# Autodesk Inventor assembly: Flysky FS-iA6 Receiver
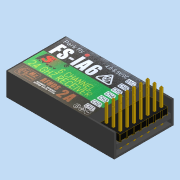
[picture p0: Inventor's stored thumbnail of the model, 180x180]
Saved by Autodesk Inventor 2022.3 (Build 263350030, 350C)
## iProperties
Created: 2022-09-05
Part Number: Flysky FS-iA6 Receiver
Document SubType Name: Assembly
Designer: admin
Author: admin
## Documents named in this file (3)
- C:\OneDrive\OneDrive - Personal\OneDrive\Documents\Inventor\BattleBot\Flysky FS-iA6 Receiver.iam
- C:\OneDrive\OneDrive - Personal\OneDrive\Documents\Inventor\BattleBot\Flysky FS-iA6 Receiver Body.ipt
- C:\OneDrive\OneDrive - Personal\OneDrive\Documents\Inventor\BattleBot\3x7 Header.ipt
## Components (2 placed, 2 different names)
1. Flysky FS-iA6 Receiver Body:1 — Rigid:1
2. 3x7 Header:1 — Rigid:1
## Relationships (1: WeldJoint 1)
- Rigid:1 [WeldJoint] (0.5 mm): Flysky FS-iA6 Receiver Body:1 ↔ 3x7 Header:1
